# Autodesk Inventor assembly: 左前脚ユニット5_MIR
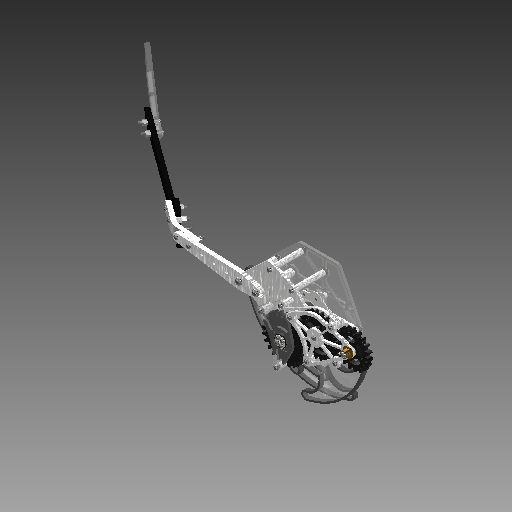
[picture p0: Inventor's stored thumbnail of the model, 512x512]
Saved by Autodesk Inventor 2020 (Build 240168000, 168)
## iProperties
Created: 2019-09-03
Part Number: 左前脚ユニット5_MIR
Document SubType Name: Assembly
Designer: 雪村
Mass: 297.882 g
Surface Area: 1626.23 cm^2
Volume: 130.235 cm^3
Density: 2.28727 g/cm^3
Author: 雪村
## Documents named in this file (30)
- C:\Users\white\Documents\SRDC\SRDC\Inventor_2017\2018年機体\2020年4年機体\右前脚ユニット5.iam
- C:\Users\white\Documents\SRDC\SRDC\Inventor_2017\2018年機体\2020年4年機体\脚内フレーム5_MIR1.ipt
- C:\Users\white\Documents\SRDC\SRDC\Inventor_2017\2018年機体\2020年4年機体\脚外フレーム5_MIR1.ipt
- C:\Users\white\Documents\SRDC\SRDC\Inventor_2017\2018年機体\2020年4年機体\前脚軸抑え1_MIR.ipt
- C:\Users\white\Documents\SRDC\SRDC\Inventor_2017\2018年機体\2020年4年機体\カウンター1.1.1_MIR.ipt
- C:\Users\white\Documents\SRDC\SRDC\Inventor_2017\2018年機体\2020年4年機体\カウンター1.4.1_MIR.ipt
- C:\Users\white\Documents\SRDC\SRDC\Inventor_2017\2018年機体\2020年4年機体\脚クランク1.iam
- C:\Users\white\Documents\SRDC\SRDC\Inventor_2017\2018年機体\2020年4年機体\ヘッケン＋揺動節2.iam
- C:\Users\white\Documents\SRDC\SRDC\Inventor_2017\2018年機体\パーツ\オイレスフランジ付き12142006.ipt
- C:\Users\white\Documents\SRDC\SRDC\Inventor_2017\2018年機体\パーツ\スペーサーm3,35.ipt
- C:\Users\white\Documents\SRDC\SRDC\Inventor_2017\2018年機体\2020年4年機体\歯車m2.z24.ipt
- C:\Users\white\Documents\SRDC\SRDC\Inventor_2017\2018年機体\パーツ\スペーサーm4,35.ipt
- C:\Users\white\Documents\SRDC\SRDC\Inventor_2017\2018年機体\2020年4年機体\脚最終段カム1.ipt
- C:\Users\white\Documents\SRDC\SRDC\Inventor_2017\2018年機体\2020年4年機体\カウンター1.2.1.ipt
- C:\Users\white\Documents\SRDC\SRDC\Inventor_2017\2018年機体\2020年4年機体\前脚ギアトレイン5_MIR.iam
- C:\Users\white\Documents\SRDC\SRDC\Inventor_2017\2018年機体\パーツ\オイレスフランジ付き12142003.ipt
- C:\Users\white\Documents\SRDC\SRDC\Inventor_2017\2018年機体\2020年4年機体\脚最終段カム5.ipt
- C:\Users\white\Documents\SRDC\SRDC\Inventor_2017\2018年機体\パーツ\ネジ皿m3,08.ipt
- C:\Users\white\Documents\SRDC\SRDC\Inventor_2017\2018年機体\パーツ\ネジ鍋m3,08.ipt
- C:\Users\white\Documents\SRDC\SRDC\Inventor_2017\2018年機体\パーツ\ネジ鍋m3,20.ipt
- C:\Users\white\Documents\SRDC\SRDC\Inventor_2017\2018年機体\パーツ\ネジ鍋m3,18.ipt
- C:\Users\white\Documents\SRDC\SRDC\Inventor_2017\2018年機体\パーツ\ネジ鍋m4,08.ipt
- C:\Users\white\Documents\SRDC\SRDC\Inventor_2017\2018年機体\パーツ\ネジ鍋m4,14.ipt
- C:\Users\white\Documents\SRDC\SRDC\Inventor_2017\2018年機体\パーツ\ナイロンナットm3.ipt
- C:\Users\white\Documents\SRDC\SRDC\Inventor_2017\2018年機体\alternative\カウンター3.ipt
- C:\Users\white\Documents\SRDC\SRDC\Inventor_2017\2018年機体\パーツ\スペーサーm3,6.ipt
- C:\Users\white\Documents\SRDC\SRDC\Inventor_2017\2018年機体\パーツ\ベアリングフランジ付き0610.3t.ipt
- C:\Users\white\Documents\SRDC\SRDC\Inventor_2017\2018年機体\パーツ\ワッシャー6.2,14.0.5t.ipt
- C:\Users\white\Documents\SRDC\SRDC\Inventor_2017\2018年機体\パーツ\スペーサーm3,10.ipt
- C:\Users\white\Documents\SRDC\SRDC\Inventor_2017\2018年機体\パーツ\ネジ鍋m3,16.ipt
## Components (58 placed, 29 different names)
1. 脚内フレーム5_MIR1:1 — メイト:5, 挿入:36, 挿入:11, メイト:7, 挿入:21, 挿入:22, 挿入:23, 挿入:24, 挿入:30, 挿入:40, 挿入:41, 挿入:42, 挿入:70, 挿入:73, 挿入:74, 挿入:75
2. 脚外フレーム5_MIR1:1 — 挿入:25, 挿入:31, 挿入:32, 挿入:43, 挿入:44, 挿入:45
3. 前脚軸抑え1_MIR:1 — 挿入:76, 挿入:77, 挿入:78, 挿入:79, 挿入:80
4. カウンター1.1.1_MIR:1 — メイト:5, 挿入:36, 挿入:26, 挿入:27, 挿入:33, 挿入:34, 挿入:49, 挿入:50
5. カウンター1.4.1_MIR:1 — 挿入:57, 挿入:58, 挿入:66, 挿入:67
6. 脚クランク1:1 [sub-assembly] — 挿入:13, メイト:3, 挿入:72
7. ヘッケン＋揺動節2:1 [sub-assembly] — メイト:4, メイト:5
8. ヘッケン＋揺動節2:2 [sub-assembly] — メイト:4
9. ヘッケン＋揺動節2:3 [sub-assembly] — メイト:5, メイト:6
10. ヘッケン＋揺動節2:4 [sub-assembly] — メイト:6, メイト:7
11. オイレスフランジ付き12142006:1 — 挿入:11, 挿入:14
12. スペーサーm3,35:1 — 挿入:21
13. スペーサーm3,35:2 — 挿入:22
14. スペーサーm3,35:3 — 挿入:24, 挿入:25
15. 歯車m2.z24:1 — 挿入:12, メイト:2
16. 脚最終段カム5:1 — 挿入:36, 挿入:37, 挿入:38, 挿入:39
17. オイレスフランジ付き12142003:1
18. スペーサーm4,35:1 — 挿入:23, 挿入:31
19. 脚最終段カム1:1 — 挿入:12, メイト:2, 挿入:13, メイト:3, 挿入:14
20. カウンター1.2.1:1 — 挿入:26, 挿入:27, 挿入:51, 挿入:52, 挿入:59, 挿入:60, 挿入:62, 挿入:63
21. 前脚ギアトレイン5_MIR:1 [sub-assembly] — 挿入:30
22. ネジ皿m3,08:1 — 挿入:40
23. ネジ鍋m3,08:1 — 挿入:43
24. ネジ鍋m3,08:2 — 挿入:44
25. ネジ鍋m3,08:3 — 挿入:42
26. ネジ鍋m3,08:4 — 挿入:45
27. ネジ鍋m3,08:5 — 挿入:41
28. ネジ鍋m3,20:1 — 挿入:36
29. ネジ鍋m3,20:3 — 挿入:37
30. ネジ鍋m3,20:4 — 挿入:38
31. ネジ鍋m3,18:2 — 挿入:39
32. ネジ鍋m4,08:1 — 挿入:32
33. ネジ鍋m4,14:1 — 挿入:33
34. ネジ鍋m4,14:2 — 挿入:34
35. ネジ鍋m3,18:4 — 挿入:57
36. ネジ鍋m3,18:5 — 挿入:63
37. ネジ鍋m3,18:6 — 挿入:58
38. ネジ鍋m3,18:7 — 挿入:50
39. ネジ鍋m3,18:8 — 挿入:49
40. ネジ鍋m3,18:9 — 挿入:62
41. ナイロンナットm3:1 — 挿入:52
42. ナイロンナットm3:2 — 挿入:51
43. ナイロンナットm3:3 — 挿入:64
44. ナイロンナットm3:4 — 挿入:65
45. ナイロンナットm3:5 — 挿入:68
46. ナイロンナットm3:6 — 挿入:69
47. カウンター3:1 — 挿入:61, メイト:9, 挿入:66, 挿入:67, 挿入:68, 挿入:69
48. スペーサーm3,6:1 — 挿入:60, 挿入:61, 挿入:64
49. スペーサーm3,6:2 — 挿入:59, メイト:9, 挿入:65
50. ベアリングフランジ付き0610.3t:1 — 挿入:71
51. ワッシャー6.2,14.0.5t:1 — 挿入:71, 挿入:72
52. スペーサーm4,35:2 — 挿入:70
53. スペーサーm3,10:1 — 挿入:75, 挿入:76
54. スペーサーm3,10:2 — 挿入:74
55. スペーサーm3,10:3 — 挿入:73, 挿入:77
56. ネジ鍋m3,16:1 — 挿入:80
57. ネジ鍋m3,16:2 — 挿入:79
58. ネジ鍋m3,16:3 — 挿入:78
## Relationships (70: Insert 62, Mate 8)
- メイト:5 [Mate]: 脚内フレーム5_MIR1:1 ↔ カウンター1.1.1_MIR:1
- 挿入:36 [Insert]: 脚内フレーム5_MIR1:1 ↔ カウンター1.1.1_MIR:1
- [Insert] (0.5 mm): 脚クランク1:1 ↔ ヘッケン＋揺動節2:2
- [Insert] (0.5 mm): 脚クランク1:1 ↔ ヘッケン＋揺動節2:1
- [Insert] (0.5 mm): 脚クランク1:1 ↔ ヘッケン＋揺動節2:3
- [Insert] (0.5 mm): 脚クランク1:1 ↔ ヘッケン＋揺動節2:4
- [Insert]: 歯車m2.z24:1 ↔ 脚最終段カム5:1
- [Insert]: 歯車m2.z24:1 ↔ 脚最終段カム5:1
- [Insert]: 脚最終段カム5:1 ↔ オイレスフランジ付き12142003:1
- 挿入:11 [Insert]: 脚内フレーム5_MIR1:1 ↔ オイレスフランジ付き12142006:1
- 挿入:12 [Insert]: 歯車m2.z24:1 ↔ 脚最終段カム1:1
- メイト:2 [Mate]: 歯車m2.z24:1 ↔ 脚最終段カム1:1
- 挿入:13 [Insert]: 脚クランク1:1 ↔ 脚最終段カム1:1
- メイト:3 [Mate]: 脚クランク1:1 ↔ 脚最終段カム1:1
- 挿入:14 [Insert]: オイレスフランジ付き12142006:1 ↔ 脚最終段カム1:1
- メイト:4 [Mate]: ヘッケン＋揺動節2:1 ↔ ヘッケン＋揺動節2:2
- メイト:5 [Mate]: ヘッケン＋揺動節2:1 ↔ ヘッケン＋揺動節2:3
- メイト:6 [Mate]: ヘッケン＋揺動節2:3 ↔ ヘッケン＋揺動節2:4
- メイト:7 [Mate]: 脚内フレーム5_MIR1:1 ↔ ヘッケン＋揺動節2:4
- 挿入:21 [Insert]: 脚内フレーム5_MIR1:1 ↔ スペーサーm3,35:1
- 挿入:22 [Insert]: 脚内フレーム5_MIR1:1 ↔ スペーサーm3,35:2
- 挿入:23 [Insert]: 脚内フレーム5_MIR1:1 ↔ スペーサーm4,35:1
- 挿入:24 [Insert]: 脚内フレーム5_MIR1:1 ↔ スペーサーm3,35:3
- 挿入:25 [Insert]: 脚外フレーム5_MIR1:1 ↔ スペーサーm3,35:3
- 挿入:26 [Insert]: カウンター1.1.1_MIR:1 ↔ カウンター1.2.1:1
- 挿入:27 [Insert]: カウンター1.1.1_MIR:1 ↔ カウンター1.2.1:1
- 挿入:30 [Insert]: 脚内フレーム5_MIR1:1 ↔ 前脚ギアトレイン5_MIR:1
- 挿入:31 [Insert]: 脚外フレーム5_MIR1:1 ↔ スペーサーm4,35:1
- 挿入:32 [Insert]: 脚外フレーム5_MIR1:1 ↔ ネジ鍋m4,08:1
- 挿入:33 [Insert]: カウンター1.1.1_MIR:1 ↔ ネジ鍋m4,14:1
- 挿入:34 [Insert]: カウンター1.1.1_MIR:1 ↔ ネジ鍋m4,14:2
- 挿入:36 [Insert]: 脚最終段カム5:1 ↔ ネジ鍋m3,20:1
- 挿入:37 [Insert]: 脚最終段カム5:1 ↔ ネジ鍋m3,20:3
- 挿入:38 [Insert]: 脚最終段カム5:1 ↔ ネジ鍋m3,20:4
- 挿入:39 [Insert]: 脚最終段カム5:1 ↔ ネジ鍋m3,18:2
- 挿入:40 [Insert]: 脚内フレーム5_MIR1:1 ↔ ネジ皿m3,08:1
- 挿入:41 [Insert]: 脚内フレーム5_MIR1:1 ↔ ネジ鍋m3,08:5
- 挿入:42 [Insert]: 脚内フレーム5_MIR1:1 ↔ ネジ鍋m3,08:3
- 挿入:43 [Insert]: 脚外フレーム5_MIR1:1 ↔ ネジ鍋m3,08:1
- 挿入:44 [Insert]: 脚外フレーム5_MIR1:1 ↔ ネジ鍋m3,08:2
- 挿入:45 [Insert]: 脚外フレーム5_MIR1:1 ↔ ネジ鍋m3,08:4
- 挿入:49 [Insert]: カウンター1.1.1_MIR:1 ↔ ネジ鍋m3,18:8
- 挿入:50 [Insert]: カウンター1.1.1_MIR:1 ↔ ネジ鍋m3,18:7
- 挿入:51 [Insert]: カウンター1.2.1:1 ↔ ナイロンナットm3:2
- 挿入:52 [Insert]: カウンター1.2.1:1 ↔ ナイロンナットm3:1
- 挿入:57 [Insert]: カウンター1.4.1_MIR:1 ↔ ネジ鍋m3,18:4
- 挿入:58 [Insert]: カウンター1.4.1_MIR:1 ↔ ネジ鍋m3,18:6
- 挿入:59 [Insert]: カウンター1.2.1:1 ↔ スペーサーm3,6:2
- 挿入:60 [Insert]: カウンター1.2.1:1 ↔ スペーサーm3,6:1
- 挿入:61 [Insert]: カウンター3:1 ↔ スペーサーm3,6:1
- メイト:9 [Mate]: カウンター3:1 ↔ スペーサーm3,6:2
- 挿入:62 [Insert]: カウンター1.2.1:1 ↔ ネジ鍋m3,18:9
- 挿入:63 [Insert]: カウンター1.2.1:1 ↔ ネジ鍋m3,18:5
- 挿入:64 [Insert]: ナイロンナットm3:3 ↔ スペーサーm3,6:1
- 挿入:65 [Insert]: ナイロンナットm3:4 ↔ スペーサーm3,6:2
- 挿入:66 [Insert]: カウンター1.4.1_MIR:1 ↔ カウンター3:1
- 挿入:67 [Insert]: カウンター1.4.1_MIR:1 ↔ カウンター3:1
- 挿入:68 [Insert]: ナイロンナットm3:5 ↔ カウンター3:1
- 挿入:69 [Insert]: ナイロンナットm3:6 ↔ カウンター3:1
- 挿入:70 [Insert]: 脚内フレーム5_MIR1:1 ↔ スペーサーm4,35:2
- 挿入:71 [Insert]: ベアリングフランジ付き0610.3t:1 ↔ ワッシャー6.2,14.0.5t:1
- 挿入:72 [Insert]: 脚クランク1:1 ↔ ワッシャー6.2,14.0.5t:1
- 挿入:73 [Insert]: 脚内フレーム5_MIR1:1 ↔ スペーサーm3,10:3
- 挿入:74 [Insert]: 脚内フレーム5_MIR1:1 ↔ スペーサーm3,10:2
- 挿入:75 [Insert]: 脚内フレーム5_MIR1:1 ↔ スペーサーm3,10:1
- 挿入:76 [Insert]: 前脚軸抑え1_MIR:1 ↔ スペーサーm3,10:1
- 挿入:77 [Insert]: 前脚軸抑え1_MIR:1 ↔ スペーサーm3,10:3
- 挿入:78 [Insert]: 前脚軸抑え1_MIR:1 ↔ ネジ鍋m3,16:3
- 挿入:79 [Insert]: 前脚軸抑え1_MIR:1 ↔ ネジ鍋m3,16:2
- 挿入:80 [Insert]: 前脚軸抑え1_MIR:1 ↔ ネジ鍋m3,16:1
